# Autodesk Inventor assembly: Carburetor
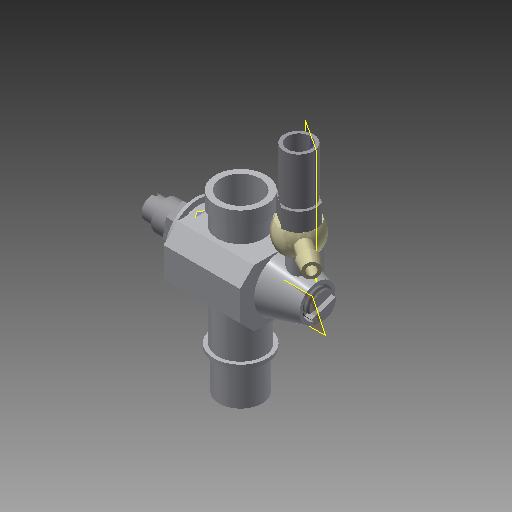
[picture p0: Inventor's stored thumbnail of the model, 512x512]
Saved by Autodesk Inventor 2017 (Build 210142000, 142)
## iProperties
Created: 2012-08-25
Part Number: Carburetor
Document SubType Name: Assembly
Designer: John
Author: John
## Documents named in this file (8)
- C:\Users\John Helfen\Videos\Inventor Presentations\Exercise Files\01_Presentations\01_01\Carburetor.iam
- C:\Users\John Helfen\Videos\Inventor Presentations\Exercise Files\01_Presentations\01_01\Gas Regulator.ipt
- C:\Users\John Helfen\Videos\Inventor Presentations\Exercise Files\01_Presentations\01_01\Mixture Control.ipt
- C:\Users\John Helfen\Videos\Inventor Presentations\Exercise Files\01_Presentations\01_01\Air Adjuster.ipt
- C:\Users\John Helfen\Videos\Inventor Presentations\Exercise Files\01_Presentations\01_01\Hex Cap.ipt
- C:\Users\John Helfen\Videos\Inventor Presentations\Exercise Files\01_Presentations\01_01\Fuel Intake.ipt
- C:\Users\John Helfen\Videos\Inventor Presentations\Exercise Files\01_Presentations\01_01\Fuel Adjuster.ipt
- C:\Users\John Helfen\Videos\Inventor Presentations\Exercise Files\01_Presentations\01_01\Carburetor Housing_v3.ipt
## Components (7 placed, 7 different names)
1. Carburetor Housing_v3:2 — Mate:6, Mate:7, Mate:10, Flush:1, Flush:2
2. Gas Regulator:1 — Mate:6, Flush:1
3. Mixture Control:1 — Flush:2
4. Air Adjuster:1
5. Hex Cap:1
6. Fuel Intake:1 — Mate:8, Mate:9, Mate:10
7. Fuel Adjuster:1 — Mate:7, Mate:8, Mate:9
## Relationships (12: Mate 10, Flush 2)
- [Mate]: Gas Regulator:1 ↔ Mixture Control:1
- [Mate]: Mixture Control:1 ↔ Air Adjuster:1
- [Mate]: Mixture Control:1 ↔ Hex Cap:1
- [Mate]: Mixture Control:1 ↔ Hex Cap:1
- [Mate] (3.175 mm): Mixture Control:1 ↔ Air Adjuster:1
- Mate:6: Carburetor Housing_v3:2 ↔ Gas Regulator:1
- Mate:7: Carburetor Housing_v3:2 ↔ Fuel Adjuster:1
- Mate:8: Fuel Intake:1 ↔ Fuel Adjuster:1
- Mate:9: Fuel Intake:1 ↔ Fuel Adjuster:1
- Mate:10: Carburetor Housing_v3:2 ↔ Fuel Intake:1
- Flush:1 (-1.27 mm): Carburetor Housing_v3:2 ↔ Gas Regulator:1
- Flush:2: Carburetor Housing_v3:2 ↔ Mixture Control:1
